# Autodesk Inventor assembly: s-assy-shooter_motor
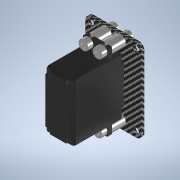
[picture p0: Inventor's stored thumbnail of the model, 180x180]
Saved by Autodesk Inventor 2022 (Build 260153000, 153)
## iProperties
Created: 2021-08-27
Part Number: s-assy-shooter_motor
Document SubType Name: Assembly
Designer: Yuta Kage
Author: Yuta Kage
## Documents named in this file (6)
- C:\Users\yuto6\Box\Public_Share\キャチロボバトルコンテスト2021\CAD\catchrobo_hardware\assy-shooter\s-assy-shooter_motor2.iam
- C:\Users\yuto6\Box\Public_Share\キャチロボバトルコンテスト2021\CAD\catchrobo_hardware\assy-robot\MG_996R.iam
- C:\Users\yuto6\Box\Public_Share\キャチロボバトルコンテスト2021\CAD\catchrobo_hardware\assy-robot\ARF-410E.ipt
- C:\Users\yuto6\Box\Public_Share\キャチロボバトルコンテスト2021\CAD\catchrobo_hardware\assy-robot\CB4-6.ipt
- C:\Users\yuto6\Box\Public_Share\キャチロボバトルコンテスト2021\CAD\catchrobo_hardware\assy-robot\CBSTSR4-6.ipt
- C:\Users\yuto6\Box\Public_Share\キャチロボバトルコンテスト2021\CAD\catchrobo_hardware\assy-shooter\s_carbon_plate4_2.ipt
## Components (14 placed, 5 different names)
1. MG_996R:1 [sub-assembly] — メイト:22, メイト:24, メイト:25, メイト:35, メイト:50, メイト:51, メイト:52, メイト:53, メイト:54, メイト:55, メイト:56, メイト:57
2. ARF-410E:2 — メイト:22, メイト:58, メイト:60
3. ARF-410E:3 — メイト:24, メイト:25
4. ARF-410E:4
5. ARF-410E:5 — メイト:35, メイト:59
6. CBSTSR4-6:2
7. CBSTSR4-6:3
8. CB4-6:4
9. CB4-6:5
10. CB4-6:6 — メイト:50, メイト:51
11. CB4-6:7 — メイト:52, メイト:53
12. CB4-6:8 — メイト:54, メイト:55
13. CB4-6:9 — メイト:56, メイト:57
14. s_carbon_plate4_2:1 — メイト:58, メイト:59, メイト:60
## Relationships (15: Mate 15)
- メイト:22 [Mate]: MG_996R:1 ↔ ARF-410E:2
- メイト:24 [Mate]: MG_996R:1 ↔ ARF-410E:3
- メイト:25 [Mate]: MG_996R:1 ↔ ARF-410E:3
- メイト:35 [Mate]: MG_996R:1 ↔ ARF-410E:5
- メイト:50 [Mate]: MG_996R:1 ↔ CB4-6:6
- メイト:51 [Mate]: MG_996R:1 ↔ CB4-6:6
- メイト:52 [Mate]: MG_996R:1 ↔ CB4-6:7
- メイト:53 [Mate]: MG_996R:1 ↔ CB4-6:7
- メイト:54 [Mate]: MG_996R:1 ↔ CB4-6:8
- メイト:55 [Mate]: MG_996R:1 ↔ CB4-6:8
- メイト:56 [Mate]: MG_996R:1 ↔ CB4-6:9
- メイト:57 [Mate]: MG_996R:1 ↔ CB4-6:9
- メイト:58 [Mate]: ARF-410E:2 ↔ s_carbon_plate4_2:1
- メイト:59 [Mate]: ARF-410E:5 ↔ s_carbon_plate4_2:1
- メイト:60 [Mate]: ARF-410E:2 ↔ s_carbon_plate4_2:1
